# Autodesk Inventor assembly: XAxis
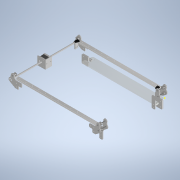
[picture p0: Inventor's stored thumbnail of the model, 180x180]
Saved by Autodesk Inventor 2022 (Build 260153000, 153)
## iProperties
Created: 2021-06-26
Part Number: XAxis
Document SubType Name: Assembly
Designer: domin
Author: domin
## Documents named in this file (17)
- C:\Users\kaebi\OneDrive - mci4me.at\03_MCI Master\4.Semester_SS2022\Masterarbeit\Software\CAD_TeachingFactory\XAxis.iam
- C:\Users\kaebi\OneDrive - mci4me.at\03_MCI Master\4.Semester_SS2022\Masterarbeit\Software\CAD_TeachingFactory\Fuehrungsschiene500mm.ipt
- C:\Users\kaebi\OneDrive - mci4me.at\03_MCI Master\4.Semester_SS2022\Masterarbeit\Software\CAD_TeachingFactory\KettenBlech_Oben.ipt
- C:\Users\kaebi\OneDrive - mci4me.at\03_MCI Master\4.Semester_SS2022\Masterarbeit\Software\CAD_TeachingFactory\Kettenblech_zusatz.ipt
- C:\Users\kaebi\OneDrive - mci4me.at\03_MCI Master\4.Semester_SS2022\Masterarbeit\Software\CAD_TeachingFactory\KettenBlech_Oben_Hinten.ipt
- C:\Users\kaebi\OneDrive - mci4me.at\03_MCI Master\4.Semester_SS2022\Masterarbeit\Software\CAD_TeachingFactory\Kettenblech_stange.ipt
- C:\Users\kaebi\OneDrive - mci4me.at\03_MCI Master\4.Semester_SS2022\Masterarbeit\Software\CAD_TeachingFactory\stange_5mm_25mm.ipt
- C:\Users\kaebi\OneDrive - mci4me.at\03_MCI Master\4.Semester_SS2022\Masterarbeit\Software\CAD_TeachingFactory\Y-Achse.ipt
- C:\Users\kaebi\OneDrive - mci4me.at\03_MCI Master\4.Semester_SS2022\Masterarbeit\Software\CAD_TeachingFactory\Y-Achse_Aufnahme_Motor.ipt
- C:\Users\kaebi\OneDrive - mci4me.at\03_MCI Master\4.Semester_SS2022\Masterarbeit\Software\CAD_TeachingFactory\Ender_Motor.ipt
- C:\Users\kaebi\OneDrive - mci4me.at\03_MCI Master\4.Semester_SS2022\Masterarbeit\Software\CAD_TeachingFactory\Umlenkrolle.ipt
- C:\Users\kaebi\OneDrive - mci4me.at\03_MCI Master\4.Semester_SS2022\Masterarbeit\Software\CAD_TeachingFactory\Umlenkrolle_5mm.ipt
- C:\Users\kaebi\OneDrive - mci4me.at\03_MCI Master\4.Semester_SS2022\Masterarbeit\Software\CAD_TeachingFactory\Endstop_holer_X.ipt
- C:\Users\kaebi\OneDrive - mci4me.at\03_MCI Master\4.Semester_SS2022\Masterarbeit\Software\CAD_TeachingFactory\Endstop.ipt
- C:\Users\kaebi\OneDrive - mci4me.at\03_MCI Master\4.Semester_SS2022\Masterarbeit\Software\CAD_TeachingFactory\Part147.ipt
- C:\Users\kaebi\OneDrive - mci4me.at\03_MCI Master\4.Semester_SS2022\Masterarbeit\Software\CAD_TeachingFactory\X_Kettenhalter.ipt
- C:\Users\kaebi\OneDrive - mci4me.at\03_MCI Master\4.Semester_SS2022\Masterarbeit\Software\CAD_TeachingFactory\Part148.ipt
## Components (34 placed, 16 different names)
1. Fuehrungsschiene500mm:1 — Mate:17, Mate:89, Mate:18, Flush:43, Flush:46, Flush:44, Flush:45, Mate:62, Flush:42, Mate:63, Flush:41, Mate:60, Mate:61, Mate:81, Mate:40, Mate:84, Mate:85, Mate:27, Mate:23, Mate:24, Mate:87, Mate:21, Flush:25, Flush:74
2. Fuehrungsschiene500mm:2 — Mate:19, Mate:88, Flush:74, Mate:82, Mate:83, Mate:28, Mate:25, Mate:26, Mate:86, Mate:22, Flush:26
3. KettenBlech_Oben:1 — Mate:87, Mate:21, Flush:25, Flush:27, Mate:29, Mate:30, Flush:33, Flush:34, Mate:56, Mate:57, Mate:74, Flush:73
4. KettenBlech_Oben:2 — Mate:86, Mate:22, Flush:26, Flush:28, Flush:35, Flush:36, Mate:58, Mate:59
5. Kettenblech_zusatz:1 — Mate:23, Mate:24, Flush:27
6. Kettenblech_zusatz:2 — Mate:25, Mate:26, Flush:28, Mate:31, Mate:32
7. KettenBlech_Oben_Hinten:1 — Mate:84, Mate:85, Mate:27, Mate:33, Flush:37, Mate:35, Mate:41, Mate:46, Mate:54, Flush:72
8. KettenBlech_Oben_Hinten:2 — Mate:82, Mate:83, Mate:28, Mate:34, Flush:38, Flush:39, Mate:47, Mate:55
9. Kettenblech_stange:1 — Mate:29, Flush:33, Mate:50
10. Kettenblech_stange:2 — Mate:30, Flush:34, Mate:52
11. Kettenblech_stange:3 — Mate:31, Flush:36, Mate:51
12. Kettenblech_stange:4 — Mate:32, Flush:35, Mate:53
13. stange_5mm_25mm:1 — Mate:33, Flush:37, Mate:48
14. stange_5mm_25mm:2 — Mate:34, Flush:38, Mate:49
15. Y-Achse:1 — Mate:35, Flush:39, Mate:42, Mate:44, Mate:45
16. Y-Achse_Aufnahme_Motor:1 — Mate:81, Mate:40, Mate:41, Angle:1, Mate:43
17. Ender_Motor:1 — Mate:42, Angle:1, Mate:43
18. Umlenkrolle:1 — Mate:44, Mate:46
19. Umlenkrolle:2 — Mate:45, Mate:47
20. Umlenkrolle_5mm:1 — Mate:48, Mate:54
21. Umlenkrolle_5mm:2 — Mate:49, Mate:55
22. Umlenkrolle_5mm:3 — Mate:50, Mate:56
23. Umlenkrolle_5mm:4 — Mate:51, Mate:58
24. Umlenkrolle_5mm:5 — Mate:52, Mate:57
25. Umlenkrolle_5mm:6 — Mate:53, Mate:59
26. Endstop_holer_X:1 — Flush:41, Mate:60, Mate:61, Mate:64, Mate:65, Mate:66
27. Endstop_holer_X:2 — Mate:62, Flush:42, Mate:63, Mate:67, Mate:68, Mate:69
28. Endstop:1 — Mate:64, Mate:65, Mate:66
29. Endstop:2 — Mate:67, Mate:68, Mate:69
30. Part147:1 — Flush:73, Flush:44, Flush:45, Mate:72, Mate:73, Mate:75
31. Part147:2 — Flush:72, Flush:43, Flush:46, Mate:78
32. X_Kettenhalter:1 — Mate:72, Mate:73, Mate:74, Mate:76, Mate:77, Mate:79, Mate:80
33. Part148:1 — Mate:75, Mate:76, Mate:77
34. Part148:2 — Mate:78, Mate:79, Mate:80
## Relationships (87: Mate 66, Flush 20, Angle 1)
- Mate:17 (420 mm): Fuehrungsschiene500mm:1
- Mate:89 (-490 mm): Fuehrungsschiene500mm:1
- Mate:18 (10 mm): Fuehrungsschiene500mm:1
- Mate:19 (420 mm): Fuehrungsschiene500mm:2
- Mate:88 (-490 mm): Fuehrungsschiene500mm:2
- Flush:74 (-390 mm): Fuehrungsschiene500mm:1 ↔ Fuehrungsschiene500mm:2
- Mate:87 (10 mm): Fuehrungsschiene500mm:1 ↔ KettenBlech_Oben:1
- Mate:86 (10 mm): Fuehrungsschiene500mm:2 ↔ KettenBlech_Oben:2
- Mate:21 (2.5 mm): Fuehrungsschiene500mm:1 ↔ KettenBlech_Oben:1
- Mate:22 (2.5 mm): Fuehrungsschiene500mm:2 ↔ KettenBlech_Oben:2
- Flush:25 (10 mm): Fuehrungsschiene500mm:1 ↔ KettenBlech_Oben:1
- Flush:26 (10 mm): Fuehrungsschiene500mm:2 ↔ KettenBlech_Oben:2
- Mate:23 (23 mm): Fuehrungsschiene500mm:1 ↔ Kettenblech_zusatz:1
- Mate:24 (22.5 mm): Fuehrungsschiene500mm:1 ↔ Kettenblech_zusatz:1
- Flush:27: KettenBlech_Oben:1 ↔ Kettenblech_zusatz:1
- Mate:25 (23 mm): Fuehrungsschiene500mm:2 ↔ Kettenblech_zusatz:2
- Mate:26 (22.5 mm): Fuehrungsschiene500mm:2 ↔ Kettenblech_zusatz:2
- Flush:28: KettenBlech_Oben:2 ↔ Kettenblech_zusatz:2
- Mate:84 (10 mm): Fuehrungsschiene500mm:1 ↔ KettenBlech_Oben_Hinten:1
- Mate:82 (10 mm): Fuehrungsschiene500mm:2 ↔ KettenBlech_Oben_Hinten:2
- Mate:85 (-10 mm): Fuehrungsschiene500mm:1 ↔ KettenBlech_Oben_Hinten:1
- Mate:83 (-10 mm): Fuehrungsschiene500mm:2 ↔ KettenBlech_Oben_Hinten:2
- Mate:27 (2.5 mm): Fuehrungsschiene500mm:1 ↔ KettenBlech_Oben_Hinten:1
- Mate:28 (2.5 mm): Fuehrungsschiene500mm:2 ↔ KettenBlech_Oben_Hinten:2
- Mate:29: KettenBlech_Oben:1 ↔ Kettenblech_stange:1
- Mate:30: KettenBlech_Oben:1 ↔ Kettenblech_stange:2
- Mate:31: Kettenblech_zusatz:2 ↔ Kettenblech_stange:3
- Mate:32: Kettenblech_zusatz:2 ↔ Kettenblech_stange:4
- Flush:33 (-6.5 mm): KettenBlech_Oben:1 ↔ Kettenblech_stange:1
- Flush:34 (-6.5 mm): KettenBlech_Oben:1 ↔ Kettenblech_stange:2
- Flush:35 (-6.5 mm): KettenBlech_Oben:2 ↔ Kettenblech_stange:4
- Flush:36 (-6.5 mm): KettenBlech_Oben:2 ↔ Kettenblech_stange:3
- Mate:33: KettenBlech_Oben_Hinten:1 ↔ stange_5mm_25mm:1
- Mate:34: KettenBlech_Oben_Hinten:2 ↔ stange_5mm_25mm:2
- Flush:37 (-6 mm): KettenBlech_Oben_Hinten:1 ↔ stange_5mm_25mm:1
- Flush:38 (-6 mm): KettenBlech_Oben_Hinten:2 ↔ stange_5mm_25mm:2
- Mate:35: KettenBlech_Oben_Hinten:1 ↔ Y-Achse:1
- Flush:39 (-1 mm): KettenBlech_Oben_Hinten:2 ↔ Y-Achse:1
- Mate:81 (10 mm): Fuehrungsschiene500mm:1 ↔ Y-Achse_Aufnahme_Motor:1
- Mate:40: Fuehrungsschiene500mm:1 ↔ Y-Achse_Aufnahme_Motor:1
- Mate:41 (192 mm): KettenBlech_Oben_Hinten:1 ↔ Y-Achse_Aufnahme_Motor:1
- Mate:42: Y-Achse:1 ↔ Ender_Motor:1
- Angle:1 (0 deg): Y-Achse_Aufnahme_Motor:1 ↔ Ender_Motor:1
- Mate:43: Y-Achse_Aufnahme_Motor:1 ↔ Ender_Motor:1
- Mate:44: Y-Achse:1 ↔ Umlenkrolle:1
- Mate:45: Y-Achse:1 ↔ Umlenkrolle:2
- Mate:46 (6 mm): KettenBlech_Oben_Hinten:1 ↔ Umlenkrolle:1
- Mate:47 (6 mm): KettenBlech_Oben_Hinten:2 ↔ Umlenkrolle:2
- Mate:48: stange_5mm_25mm:1 ↔ Umlenkrolle_5mm:1
- Mate:49: stange_5mm_25mm:2 ↔ Umlenkrolle_5mm:2
- Mate:50: Kettenblech_stange:1 ↔ Umlenkrolle_5mm:3
- Mate:51: Kettenblech_stange:3 ↔ Umlenkrolle_5mm:4
- Mate:52: Kettenblech_stange:2 ↔ Umlenkrolle_5mm:5
- Mate:53: Kettenblech_stange:4 ↔ Umlenkrolle_5mm:6
- Mate:54 (5.5 mm): KettenBlech_Oben_Hinten:1 ↔ Umlenkrolle_5mm:1
- Mate:55 (5.5 mm): KettenBlech_Oben_Hinten:2 ↔ Umlenkrolle_5mm:2
- Mate:56 (5.5 mm): KettenBlech_Oben:1 ↔ Umlenkrolle_5mm:3
- Mate:57 (5.5 mm): KettenBlech_Oben:1 ↔ Umlenkrolle_5mm:5
- Mate:58 (5.5 mm): KettenBlech_Oben:2 ↔ Umlenkrolle_5mm:4
- Mate:59 (5.5 mm): KettenBlech_Oben:2 ↔ Umlenkrolle_5mm:6
- Flush:41 (-20 mm): Fuehrungsschiene500mm:1 ↔ Endstop_holer_X:1
- Mate:60: Fuehrungsschiene500mm:1 ↔ Endstop_holer_X:1
- Mate:61 (2.5 mm): Fuehrungsschiene500mm:1 ↔ Endstop_holer_X:1
- Mate:62: Fuehrungsschiene500mm:1 ↔ Endstop_holer_X:2
- Flush:42 (-20 mm): Fuehrungsschiene500mm:1 ↔ Endstop_holer_X:2
- Mate:63 (2.5 mm): Fuehrungsschiene500mm:1 ↔ Endstop_holer_X:2
- Mate:64: Endstop_holer_X:1 ↔ Endstop:1
- Mate:65: Endstop_holer_X:1 ↔ Endstop:1
- Mate:66: Endstop_holer_X:1 ↔ Endstop:1
- Mate:67: Endstop_holer_X:2 ↔ Endstop:2
- Mate:68: Endstop_holer_X:2 ↔ Endstop:2
- Mate:69: Endstop_holer_X:2 ↔ Endstop:2
- Flush:73: KettenBlech_Oben:1 ↔ Part147:1
- Flush:72: KettenBlech_Oben_Hinten:1 ↔ Part147:2
- Flush:43: Fuehrungsschiene500mm:1 ↔ Part147:2
- Flush:44: Fuehrungsschiene500mm:1 ↔ Part147:1
- Flush:45 (-85 mm): Fuehrungsschiene500mm:1 ↔ Part147:1
- Flush:46 (-85 mm): Fuehrungsschiene500mm:1 ↔ Part147:2
- Mate:72: Part147:1 ↔ X_Kettenhalter:1
- Mate:73: Part147:1 ↔ X_Kettenhalter:1
- Mate:74: KettenBlech_Oben:1 ↔ X_Kettenhalter:1
- Mate:75: Part147:1 ↔ Part148:1
- Mate:76: X_Kettenhalter:1 ↔ Part148:1
- Mate:77: X_Kettenhalter:1 ↔ Part148:1
- Mate:78: Part147:2 ↔ Part148:2
- Mate:79: X_Kettenhalter:1 ↔ Part148:2
- Mate:80: X_Kettenhalter:1 ↔ Part148:2
